# Autodesk Inventor assembly: controller
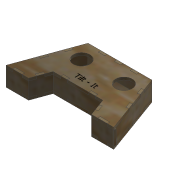
[picture p0: Inventor's stored thumbnail of the model, 180x180]
Saved by Autodesk Inventor 2016 (Build 200138000, 138)
## iProperties
Created: 2015-10-06
Part Number: controller
Document SubType Name: Assembly
Designer: Haukur
Author: Haukur
## Documents named in this file (8)
- C:\Users\Stefan\Documents\t-411-mech-2015\group\TiltIt\kit\controller\controller.iam
- C:\Users\Stefan\Documents\t-411-mech-2015\group\TiltIt\kit\controller\back.ipt
- C:\Users\Stefan\Documents\t-411-mech-2015\group\TiltIt\kit\controller\front(vga).ipt
- C:\Users\Stefan\Documents\t-411-mech-2015\group\TiltIt\kit\controller\hlid.ipt
- C:\Users\Stefan\Documents\t-411-mech-2015\group\TiltIt\kit\controller\stubbur.ipt
- C:\Users\Stefan\Documents\t-411-mech-2015\group\TiltIt\kit\controller\innanverdurstubbur.ipt
- C:\Users\Stefan\Documents\t-411-mech-2015\group\TiltIt\kit\controller\front(magi).ipt
- C:\Users\Stefan\Documents\t-411-mech-2015\group\TiltIt\kit\controller\top.ipt
## Components (10 placed, 7 different names)
1. back:1 — Mate:1, Mate:2, Mate:3, Mate:10, Mate:11, Mate:12, Mate:13, Mate:14, Mate:15, Mate:16, Mate:17, Mate:18, Mate:19, Mate:20, Mate:21, Mate:22, Mate:23, Mate:24, Mate:30, Mate:32, Flush:2, Mate:33, Mate:34, Flush:3, Mate:35
2. front(vga):1 — Mate:1, Mate:2, Mate:3, Mate:31
3. stubbur:1 — Mate:13, Mate:14, Mate:15, Flush:1
4. stubbur:2 — Mate:10, Mate:11, Mate:12
5. innanverdurstubbur:1 — Mate:16, Mate:17, Mate:18
6. innanverdurstubbur:2 — Mate:19, Mate:20, Mate:21, Mate:36
7. front(magi):1 — Mate:22, Mate:23, Mate:24
8. hlid:1 — Mate:32, Flush:2, Mate:33
9. hlid:2 — Mate:30, Mate:34, Flush:3, Mate:35
10. top:1 — Mate:31, Flush:1, Mate:36
## Relationships (28: Mate 25, Flush 3)
- Mate:1: back:1 ↔ front(vga):1
- Mate:2: back:1 ↔ front(vga):1
- Mate:3: back:1 ↔ front(vga):1
- Mate:10: back:1 ↔ stubbur:2
- Mate:11: back:1 ↔ stubbur:2
- Mate:12: back:1 ↔ stubbur:2
- Mate:13: back:1 ↔ stubbur:1
- Mate:14: back:1 ↔ stubbur:1
- Mate:15: back:1 ↔ stubbur:1
- Mate:16: back:1 ↔ innanverdurstubbur:1
- Mate:17: back:1 ↔ innanverdurstubbur:1
- Mate:18: back:1 ↔ innanverdurstubbur:1
- Mate:19: back:1 ↔ innanverdurstubbur:2
- Mate:20: back:1 ↔ innanverdurstubbur:2
- Mate:21: back:1 ↔ innanverdurstubbur:2
- Mate:22: back:1 ↔ front(magi):1
- Mate:23: back:1 ↔ front(magi):1
- Mate:24: back:1 ↔ front(magi):1
- Mate:30: back:1 ↔ hlid:2
- Mate:31: front(vga):1 ↔ top:1
- Flush:1: stubbur:1 ↔ top:1
- Mate:32: back:1 ↔ hlid:1
- Flush:2: back:1 ↔ hlid:1
- Mate:33: back:1 ↔ hlid:1
- Mate:34: back:1 ↔ hlid:2
- Flush:3: back:1 ↔ hlid:2
- Mate:35: back:1 ↔ hlid:2
- Mate:36: innanverdurstubbur:2 ↔ top:1
